# Autodesk Inventor assembly: Assembly_Cube_v4_xystage_diamond
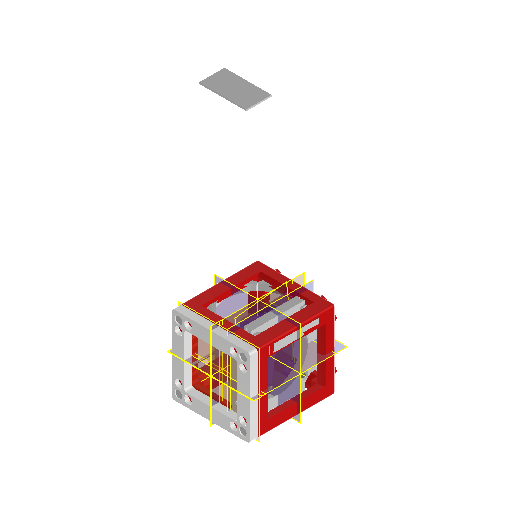
[picture p0: Inventor's stored thumbnail of the model, 512x512]
Saved by Autodesk Inventor 2025.1 (Build 291241020, 241B)
## iProperties
Created: 2024-10-03
Part Number: Assembly_Cube_v4_xystage_diamond
Document SubType Name: Assembly
Designer: diederichbenedict
Author: diederichbenedict
## Documents named in this file (8)
- C:\Users\diederichbenedict\Dropbox\Dokumente\Promotion\PROJECTS\TechnicalDocs-openUC2-QBox\Production_Files\CAD_Files\INVENTOR\Assembly_Cube_v4_xystage_diamond.iam
- C:\Users\diederichbenedict\Dropbox\Dokumente\Promotion\PROJECTS\TechnicalDocs-openUC2-QBox\Production_Files\CAD_Files\INVENTOR\Assembly_Cube_v4.iam
- C:\Users\diederichbenedict\Dropbox\Dokumente\Promotion\PROJECTS\TechnicalDocs-openUC2-QBox\Production_Files\CAD_Files\INVENTOR\10_Insert_v4.ipt
- C:\Users\diederichbenedict\Dropbox\Dokumente\Promotion\PROJECTS\TechnicalDocs-openUC2-QBox\Production_Files\CAD_Files\INVENTOR\20_Cube_4_insert_xy_slider.ipt
- C:\Users\diederichbenedict\Documents\Inventor\Content Center Files\R2025\en-US\DIN 912\DIN 912 - M3 x 0.5 x 8 x 6.75.ipt
- C:\Users\diederichbenedict\Dropbox\Dokumente\Promotion\PROJECTS\TechnicalDocs-openUC2-QBox\Production_Files\CAD_Files\INVENTOR\20_Cube_4_insert_xy_levelarm.ipt
- C:\Users\diederichbenedict\Dropbox\Dokumente\Promotion\PROJECTS\TechnicalDocs-openUC2-QBox\Production_Files\CAD_Files\INVENTOR\20_Cube_4_insert_xy_levelarm_2.ipt
- C:\Users\diederichbenedict\Dropbox\Dokumente\Promotion\PROJECTS\TechnicalDocs-openUC2-QBox\Production_Files\CAD_Files\INVENTOR\00_Antenna_dummy.ipt
## Components (12 placed, 7 different names)
1. Assembly_Cube_v4:1 [sub-assembly] — Mate:1, Mate:2, Mate:5, Angle:1
2. 10_Insert_v4:1 — Mate:5, Angle:1, Insert:1, Insert:2, Insert:3, Insert:4, Mate:6
3. DIN 912 - replaced by DIN EN ISO 4762 M3 x 8:1 — Insert:2, Tangent:3
4. DIN 912 - replaced by DIN EN ISO 4762 M3 x 8:2 — Insert:3, Tangent:2
5. DIN 912 - replaced by DIN EN ISO 4762 M3 x 8:3 — Insert:8
6. DIN 912 - replaced by DIN EN ISO 4762 M3 x 8:4 — Insert:4, Tangent:1
7. DIN 912 - replaced by DIN EN ISO 4762 M3 x 8:5 — Insert:1
8. DIN 912 - replaced by DIN EN ISO 4762 M3 x 8:6 — Insert:9, Insert:10
9. 20_Cube_4_insert_xy_slider:1 — Tangent:1, Tangent:2, Mate:6, Insert:7, Insert:10
10. 20_Cube_4_insert_xy_levelarm:1 — Insert:7, Tangent:3, Insert:8
11. 20_Cube_4_insert_xy_levelarm_2:1 — Insert:9
12. 00_Antenna_dummy:1
## Relationships (16: Insert 8, Mate 4, Tangent 3, Angle 1)
- Mate:1: Assembly_Cube_v4:1
- Mate:2: Assembly_Cube_v4:1
- Mate:5: Assembly_Cube_v4:1 ↔ 10_Insert_v4:1
- Angle:1 (180 deg): Assembly_Cube_v4:1 ↔ 10_Insert_v4:1
- Insert:1 (3 mm): 10_Insert_v4:1 ↔ DIN 912 - replaced by DIN EN ISO 4762 M3 x 8:5
- Insert:2 (3 mm): 10_Insert_v4:1 ↔ DIN 912 - replaced by DIN EN ISO 4762 M3 x 8:1
- Insert:3 (3 mm): 10_Insert_v4:1 ↔ DIN 912 - replaced by DIN EN ISO 4762 M3 x 8:2
- Insert:4 (3 mm): 10_Insert_v4:1 ↔ DIN 912 - replaced by DIN EN ISO 4762 M3 x 8:4
- Tangent:1: DIN 912 - replaced by DIN EN ISO 4762 M3 x 8:4 ↔ 20_Cube_4_insert_xy_slider:1
- Tangent:2: DIN 912 - replaced by DIN EN ISO 4762 M3 x 8:2 ↔ 20_Cube_4_insert_xy_slider:1
- Mate:6: 10_Insert_v4:1 ↔ 20_Cube_4_insert_xy_slider:1
- Insert:7: 20_Cube_4_insert_xy_slider:1 ↔ 20_Cube_4_insert_xy_levelarm:1
- Tangent:3: DIN 912 - replaced by DIN EN ISO 4762 M3 x 8:1 ↔ 20_Cube_4_insert_xy_levelarm:1
- Insert:8: DIN 912 - replaced by DIN EN ISO 4762 M3 x 8:3 ↔ 20_Cube_4_insert_xy_levelarm:1
- Insert:9: DIN 912 - replaced by DIN EN ISO 4762 M3 x 8:6 ↔ 20_Cube_4_insert_xy_levelarm_2:1
- Insert:10 (3 mm): DIN 912 - replaced by DIN EN ISO 4762 M3 x 8:6 ↔ 20_Cube_4_insert_xy_slider:1
